# Autodesk Inventor assembly: mx28_withHorn_andSchwung
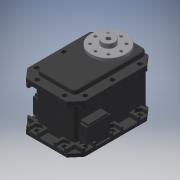
[picture p0: Inventor's stored thumbnail of the model, 180x180]
Saved by Autodesk Inventor 2016 (Build 200138000, 138)
## iProperties
Created: 2014-04-23
Part Number: mx28_withHorn_andSchwung
Document SubType Name: Assembly
Designer: BitBots
Author: BitBots
## Documents named in this file (4)
- C:\Hambot\motors\MX28\mx28_with_bearing.iam
- C:\Hambot\motors\MX28\mx28_body.ipt
- C:\Hambot\motors\MX28\HN07-N101.ipt
- C:\Hambot\motors\MX28\HN07-i101.ipt
## Components (3 placed, 3 different names)
1. mx28_body:1 — Rotational:2, Rotational:1
2. HN07-N101:1 — Rotational:2
3. HN07-i101:1 — Rotational:1
## Relationships (2: RevoluteJoint 2)
- Rotational:2 [RevoluteJoint]: mx28_body:1 ↔ HN07-N101:1
- Rotational:1 [RevoluteJoint]: mx28_body:1 ↔ HN07-i101:1
